# Autodesk Inventor assembly: Synchronous Belts Transmission
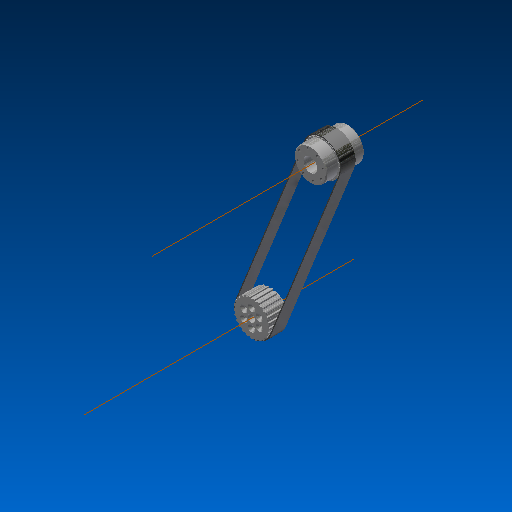
[picture p0: Inventor's stored thumbnail of the model, 512x512]
Saved by Autodesk Inventor 2018 (Build 220112000, 112)
## iProperties
Created: 2020-03-19
Part Number: Synchronous Belts Transmission
Document SubType Name: Assembly
Designer: Bunny320
ClientObjectVersion: 1
Author: Bunny320
## Documents named in this file (4)
- D:\Seerosenstr\sechs\4-CAD\generated\J3_belt\Design Accelerator\Synchronous Belts Transmission1.iam
- D:\Seerosenstr\sechs\4-CAD\generated\J3_belt\Design Accelerator\Synchronous Belt1.ipt
- D:\Seerosenstr\sechs\4-CAD\generated\J3_belt\Design Accelerator\Synchronous Pulley11.ipt
- D:\Seerosenstr\sechs\4-CAD\generated\J3_belt\Design Accelerator\Synchronous Pulley21.ipt
## Components (3 placed, 3 different names)
1. Synchronous Belt:1 — Flush:1, Mate:1, Mate:2, Flush:2, Mate:3, Mate:4
2. Synchronous Pulley1:1 — Flush:1, Mate:1, Mate:2, Rotation:1
3. Synchronous Pulley2:1 — Flush:2, Mate:3, Rotation:1, Mate:4
## Relationships (7: Mate 4, Flush 2, RelateRotation 1)
- Flush:1: Synchronous Belt:1 ↔ Synchronous Pulley1:1
- Mate:1: Synchronous Belt:1 ↔ Synchronous Pulley1:1
- Mate:2: Synchronous Belt:1 ↔ Synchronous Pulley1:1
- Flush:2: Synchronous Belt:1 ↔ Synchronous Pulley2:1
- Mate:3: Synchronous Belt:1 ↔ Synchronous Pulley2:1
- Rotation:1 [RelateRotation] (1 ul): Synchronous Pulley1:1 ↔ Synchronous Pulley2:1
- Mate:4: Synchronous Belt:1 ↔ Synchronous Pulley2:1
